# Autodesk Inventor assembly: 1444-17154_Aluminum_Chasis
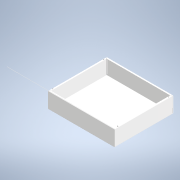
[picture p0: Inventor's stored thumbnail of the model, 180x180]
Saved by Autodesk Inventor 2021 (Build 250183000, 183)
## iProperties
Created: 2013-07-04
Part Number: 1444-17154_Aluminum_Chasis
Document SubType Name: Assembly
Designer: Admin
Sending System: Autodesk Inventor 2013
Preprocessor: Autodesk Inventor 2013
Title: E:\Eng\Customer Service\Drawings\1444 & 1434\STEP Files\Conversion\1434-1715 & 1444-17154\1444-17154.iam.stp
## Documents named in this file (4)
- C:\Users\Admin\Dropbox (MIT)\MPI Group Folder\MPS\Inventor_Parts\MPSV2\Digikey Parts\1444-17154_Aluminum_Chasis.iam
- C:\Users\Admin\Dropbox (MIT)\MPI Group Folder\MPS\Inventor_Parts\MPSV2\Digikey Parts\1444-17154.ipt
- C:\Users\Admin\Dropbox (MIT)\MPI Group Folder\MPS\Inventor_Parts\MPSV2\Digikey Parts\1434-1715.ipt
- C:\Users\Admin\Dropbox (MIT)\MPI Group Folder\MPS\Inventor_Parts\MPSV2\Digikey Parts\6-32 (SC18394).ipt
## Components (6 placed, 3 different names)
1. 1444-17154:1 — Angle:1, Mate:1, Flush:1
2. 1434-1715:1 — Angle:1, Mate:1, Flush:1
3. 6-32 (SC18394):1
4. 6-32 (SC18394):2
5. 6-32 (SC18394):3
6. 6-32 (SC18394):4
## Relationships (3: Angle 1, Mate 1, Flush 1)
- Angle:1 (135 deg): 1444-17154:1 ↔ 1434-1715:1
- Mate:1: 1444-17154:1 ↔ 1434-1715:1
- Flush:1: 1444-17154:1 ↔ 1434-1715:1
